# Autodesk Inventor assembly: EDMO_TrackStar_TS_411MG
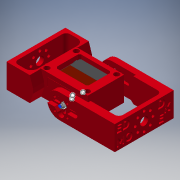
[picture p0: Inventor's stored thumbnail of the model, 180x180]
Saved by Autodesk Inventor 2019 (Build 230136000, 136)
## iProperties
Created: 2020-08-13
Part Number: EDMO_TrackStar_TS_411MG
Document SubType Name: Assembly
Designer: lucas.dahl
Author: lucas.dahl
## Documents named in this file (10)
- D:\PhD\Teaching\RES and Projects Construction\CAD_Files\EDMO_TrackStar_Module\EDMO_TrackStar_TS_411MG.iam
- D:\PhD\Teaching\RES and Projects Construction\CAD_Files\EDMO_TrackStar_Module\Trackstar_Servo_TS411MG.ipt
- C:\Users\lucas.dahl\Documents\Inventor\Content Center Files\R2019\en-US\DIN 125-1  A\DIN 125 - A 3.2.ipt
- C:\Users\lucas.dahl\Documents\Inventor\Content Center Files\R2019\en-US\DIN 985\DIN 985 - M3.ipt
- C:\Users\lucas.dahl\Documents\Inventor\Content Center Files\R2019\en-US\DIN 912\DIN 912 - M3 x 0.5 x 16 x 14.75.ipt
- C:\Users\lucas.dahl\Documents\Inventor\Content Center Files\R2019\en-US\DIN 934\DIN 934 - M3 x 0.5.ipt
- C:\Users\lucas.dahl\Documents\Inventor\Content Center Files\R2019\en-US\DIN 912\DIN 912 - M3 x 0.5 x 20 x 18.75.ipt
- D:\PhD\Teaching\RES and Projects Construction\CAD_Files\EDMO_TrackStar_Module\EDMO1-1_Arm.ipt
- D:\PhD\Teaching\RES and Projects Construction\CAD_Files\EDMO_TrackStar_Module\EDMO1-1_Body.ipt
- D:\PhD\Teaching\RES and Projects Construction\CAD_Files\EDMO_TrackStar_Module\EDMO1-1_Cover.ipt
## Components (18 placed, 9 different names)
1. EDMO1-1_Body:1 — Mate:1, Flush:1, Mate:2, Mate:3, Flush:2, Flush:3, Mate:5, Insert:1, Insert:2, Insert:13, Insert:14, Insert:15, Insert:16, Angle:2, Angle:3, Angle:4, Angle:5
2. Trackstar_Servo_TS411MG:1 — Mate:1, Flush:1, Mate:2, Mate:4
3. EDMO1-1_Cover:1 — Mate:3, Flush:2, Flush:3, Angle:1, Insert:9, Insert:10, Insert:11, Insert:12
4. EDMO1-1_Arm:1 — Mate:4, Mate:5, Insert:4, Angle:1
5. DIN 912 - replaced by DIN EN ISO 4762 M3 x 16:1 — Insert:1
6. DIN 125-1 A A 3.2:1 — Insert:2, Insert:5
7. DIN 125-1 A A 3.2:2 — Insert:4, Insert:7
8. DIN 934 - replaced by DIN EN 24032/28673/28674 M3:1 — Insert:8
9. DIN 912 - replaced by DIN EN ISO 4762 M3 x 20:1 — Insert:9
10. DIN 912 - replaced by DIN EN ISO 4762 M3 x 20:2 — Insert:10
11. DIN 912 - replaced by DIN EN ISO 4762 M3 x 20:3 — Insert:12
12. DIN 912 - replaced by DIN EN ISO 4762 M3 x 20:4 — Insert:11
13. DIN 985 - replaced by DIN EN ISO 10511 M3:1 — Insert:5, Insert:8
14. DIN 985 - replaced by DIN EN ISO 10511 M3:2 — Insert:7
15. DIN 985 - replaced by DIN EN ISO 10511 M3:3 — Insert:13, Angle:3
16. DIN 985 - replaced by DIN EN ISO 10511 M3:4 — Insert:14, Angle:4
17. DIN 985 - replaced by DIN EN ISO 10511 M3:5 — Insert:15, Angle:2
18. DIN 985 - replaced by DIN EN ISO 10511 M3:6 — Insert:16, Angle:5
## Relationships (27: Insert 14, Mate 5, Angle 5, Flush 3)
- Mate:1 (0.05 mm): EDMO1-1_Body:1 ↔ Trackstar_Servo_TS411MG:1
- Flush:1: EDMO1-1_Body:1 ↔ Trackstar_Servo_TS411MG:1
- Mate:2 (0.1 mm): EDMO1-1_Body:1 ↔ Trackstar_Servo_TS411MG:1
- Mate:3: EDMO1-1_Body:1 ↔ EDMO1-1_Cover:1
- Flush:2: EDMO1-1_Body:1 ↔ EDMO1-1_Cover:1
- Flush:3: EDMO1-1_Body:1 ↔ EDMO1-1_Cover:1
- Mate:4: Trackstar_Servo_TS411MG:1 ↔ EDMO1-1_Arm:1
- Mate:5: EDMO1-1_Body:1 ↔ EDMO1-1_Arm:1
- Insert:1: EDMO1-1_Body:1 ↔ DIN 912 - replaced by DIN EN ISO 4762 M3 x 16:1
- Insert:2: EDMO1-1_Body:1 ↔ DIN 125-1 A A 3.2:1
- Insert:4: EDMO1-1_Arm:1 ↔ DIN 125-1 A A 3.2:2
- Insert:5: DIN 125-1 A A 3.2:1 ↔ DIN 985 - replaced by DIN EN ISO 10511 M3:1
- Insert:7: DIN 125-1 A A 3.2:2 ↔ DIN 985 - replaced by DIN EN ISO 10511 M3:2
- Angle:1 (0 deg): EDMO1-1_Cover:1 ↔ EDMO1-1_Arm:1
- Insert:8: DIN 934 - replaced by DIN EN 24032/28673/28674 M3:1 ↔ DIN 985 - replaced by DIN EN ISO 10511 M3:1
- Insert:9: EDMO1-1_Cover:1 ↔ DIN 912 - replaced by DIN EN ISO 4762 M3 x 20:1
- Insert:10: EDMO1-1_Cover:1 ↔ DIN 912 - replaced by DIN EN ISO 4762 M3 x 20:2
- Insert:11: EDMO1-1_Cover:1 ↔ DIN 912 - replaced by DIN EN ISO 4762 M3 x 20:4
- Insert:12: EDMO1-1_Cover:1 ↔ DIN 912 - replaced by DIN EN ISO 4762 M3 x 20:3
- Insert:13: EDMO1-1_Body:1 ↔ DIN 985 - replaced by DIN EN ISO 10511 M3:3
- Insert:14: EDMO1-1_Body:1 ↔ DIN 985 - replaced by DIN EN ISO 10511 M3:4
- Insert:15: EDMO1-1_Body:1 ↔ DIN 985 - replaced by DIN EN ISO 10511 M3:5
- Insert:16: EDMO1-1_Body:1 ↔ DIN 985 - replaced by DIN EN ISO 10511 M3:6
- Angle:2 (0 deg): EDMO1-1_Body:1 ↔ DIN 985 - replaced by DIN EN ISO 10511 M3:5
- Angle:3 (0 deg): EDMO1-1_Body:1 ↔ DIN 985 - replaced by DIN EN ISO 10511 M3:3
- Angle:4 (0 deg): EDMO1-1_Body:1 ↔ DIN 985 - replaced by DIN EN ISO 10511 M3:4
- Angle:5 (0 deg): EDMO1-1_Body:1 ↔ DIN 985 - replaced by DIN EN ISO 10511 M3:6
